# Autodesk Inventor assembly: PSU
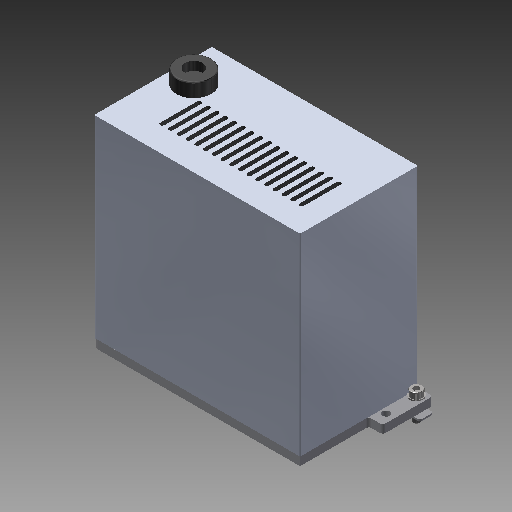
[picture p0: Inventor's stored thumbnail of the model, 512x512]
Saved by Autodesk Inventor 2018 (Build 220112000, 112)
## iProperties
Created: 2016-07-28
Part Number: PSU
Document SubType Name: Assembly
Designer: User
Author: User
## Documents named in this file (7)
- C:\Users\Dan\OneDrive\SL-Inventor\The Beast v1.2 PackandGo\Workspaces\Workspace\PSU.iam
- C:\Users\Dan\OneDrive\SL-Inventor\The Beast v1.2 PackandGo\Workspaces\Workspace\PSU Mount Hipro.ipt
- C:\Users\Dan\OneDrive\SL-Inventor\The Beast v1.2 PackandGo\Workspaces\Workspace\power supply.ipt
- C:\Users\Dan\OneDrive\SL-Inventor\The Beast v1.2 PackandGo\Workspaces\Workspace\en-US\ANSI B18.3.1M(6)\ANSI B18.3.1M - M3x0.5 x 10(1).ipt
- C:\Users\Dan\OneDrive\SL-Inventor\The Beast v1.2 PackandGo\Workspaces\Workspace\en-US\JIS B 1251 C1 (1L 1H)\JIS B 1251  - 5 1L.ipt
- C:\Users\Dan\OneDrive\SL-Inventor\The Beast v1.2 PackandGo\Workspaces\Workspace\en-US\ANSI B18.3.1M(6)\ANSI B18.3.1M - M5x0.8 x 16(1).ipt
- C:\Users\Dan\OneDrive\SL-Inventor\The Beast v1.2 PackandGo\Workspaces\Workspace\M5 Tee Nut-Generic_MIR_MIR.ipt
## Components (10 placed, 6 different names)
1. PSU Mount Hipro:1
2. power supply:1
3. M5 Tee Nut-Generic_MIR_MIR:1
4. JIS B 1251 Class 1 (1L/1H) 5 1L:1
5. Forged Socket Head Cap Screw - Metric M5x0.8 x 16:1
6. M5 Tee Nut-Generic_MIR_MIR:2
7. Forged Socket Head Cap Screw - Metric M5x0.8 x 16:2
8. JIS B 1251 Class 1 (1L/1H) 5 1L:2
9. Forged Socket Head Cap Screw - Metric M3x0.5 x 10:3
10. Forged Socket Head Cap Screw - Metric M3x0.5 x 10:4
## Relationships (9: Mate 5, Insert 3, Angle 1)
- [Mate]: PSU Mount Hipro:1 ↔ power supply:1
- [Angle] (0 deg): PSU Mount Hipro:1 ↔ power supply:1
- [Insert]: PSU Mount Hipro:1 ↔ Forged Socket Head Cap Screw - Metric M3x0.5 x 10:3
- [Insert]: PSU Mount Hipro:1 ↔ Forged Socket Head Cap Screw - Metric M3x0.5 x 10:4
- [Insert]: PSU Mount Hipro:1 ↔ JIS B 1251 Class 1 (1L/1H) 5 1L:2
- [Mate]: PSU Mount Hipro:1 ↔ Forged Socket Head Cap Screw - Metric M5x0.8 x 16:2
- [Mate] (3 mm): PSU Mount Hipro:1 ↔ M5 Tee Nut-Generic_MIR_MIR:1
- [Mate]: M5 Tee Nut-Generic_MIR_MIR:2 ↔ Forged Socket Head Cap Screw - Metric M5x0.8 x 16:2
- [Mate] (3 mm): PSU Mount Hipro:1 ↔ M5 Tee Nut-Generic_MIR_MIR:2
